# Autodesk Inventor assembly: SDA 63 50 Full
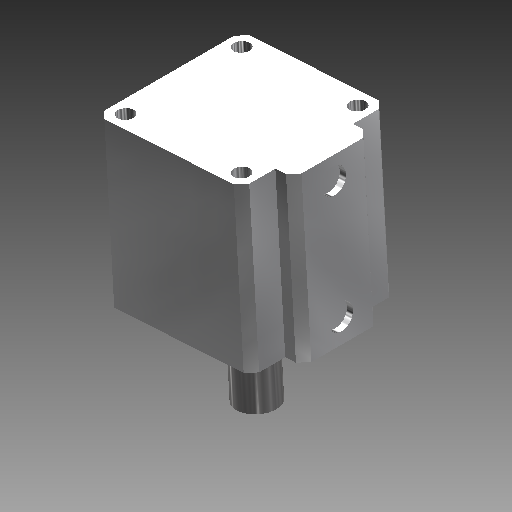
[picture p0: Inventor's stored thumbnail of the model, 512x512]
Saved by Autodesk Inventor 2019 (Build 230136000, 136)
## iProperties
Created: 2019-10-25
Part Number: SDA 63 50 Full
Document SubType Name: Assembly
Designer: Mark
Mass: 1401.99 g
Surface Area: 497.597 cm^2
Volume: 490.733 cm^3
Density: 2.85693 g/cm^3
Author: Mark
## Documents named in this file (3)
- C:\Users\Mark\Desktop\7738 Helion Engineering\7738-CAD-prep\Butterfly Drive Mk2\Butterfly Base\SDA 63 50 Full.iam
- C:\Users\Mark\Desktop\7738 Helion Engineering\7738-CAD-prep\Butterfly drive\SDA 63 50.ipt
- C:\Users\Mark\Desktop\7738 Helion Engineering\7738-CAD-prep\Butterfly drive\SDA 63 50 Stroke Full.ipt
## Components (2 placed, 2 different names)
1. SDA 63 50:1 — Mate:1, Flush:1
2. SDA 63 50 Stroke Full:1 — Mate:1, Flush:1
## Relationships (2: Mate 1, Flush 1)
- Mate:1: SDA 63 50:1 ↔ SDA 63 50 Stroke Full:1
- Flush:1 (-40 mm): SDA 63 50:1 ↔ SDA 63 50 Stroke Full:1
